# Autodesk Inventor assembly: RD-A001-P003_1
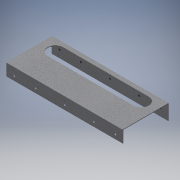
[picture p0: Inventor's stored thumbnail of the model, 180x180]
Saved by Autodesk Inventor 2017 (Build 210142000, 142)
## iProperties
Created: 2017-05-03
Part Number: RD-A001-P003_1
Document SubType Name: Assembly
Designer: krosie
Author: krosie
## Documents named in this file (3)
- C:\Users\Kathryn Rosie\Google Drive\HERA\hera-cad\Node\Concept-ICTS\ICTS-20170411\RD-A001-P003_1.iam
- C:\Users\Kathryn Rosie\Google Drive\HERA\hera-cad\Node\Concept-ICTS\ICTS-20170411\P-FHS-M6-18.ipt
- C:\Users\Kathryn Rosie\Google Drive\HERA\hera-cad\Node\20171003\SidePanelCoverSpacer.ipt
## Components (6 placed, 2 different names)
1. SidePanelCoverSpacer:1 — Mate:1, Mate:2, Mate:3, Mate:4, Mate:5, Flush:1, Flush:2, Flush:3, Flush:4, Flush:5
2. P-FHS-M6-18 — Mate:1, Flush:5
3. P-FHS-M6-18:1 — Mate:5, Flush:1
4. P-FHS-M6-18:2 — Mate:4, Flush:2
5. P-FHS-M6-18:3 — Mate:3, Flush:3
6. P-FHS-M6-18:4 — Mate:2, Flush:4
## Relationships (10: Mate 5, Flush 5)
- Mate:1: SidePanelCoverSpacer:1 ↔ P-FHS-M6-18
- Mate:2: SidePanelCoverSpacer:1 ↔ P-FHS-M6-18:4
- Mate:3: SidePanelCoverSpacer:1 ↔ P-FHS-M6-18:3
- Mate:4: SidePanelCoverSpacer:1 ↔ P-FHS-M6-18:2
- Mate:5: SidePanelCoverSpacer:1 ↔ P-FHS-M6-18:1
- Flush:1: SidePanelCoverSpacer:1 ↔ P-FHS-M6-18:1
- Flush:2: SidePanelCoverSpacer:1 ↔ P-FHS-M6-18:2
- Flush:3: SidePanelCoverSpacer:1 ↔ P-FHS-M6-18:3
- Flush:4: SidePanelCoverSpacer:1 ↔ P-FHS-M6-18:4
- Flush:5: SidePanelCoverSpacer:1 ↔ P-FHS-M6-18
